# Autodesk Inventor assembly: Кресло простое
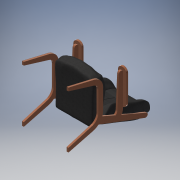
[picture p0: Inventor's stored thumbnail of the model, 180x180]
Saved by Autodesk Inventor 2019 (Build 230136000, 136)
## iProperties
Created: 2018-10-09
Part Number: Кресло простое
Material: Типовые
Document SubType Name: Assembly
Designer: Андреев Н.Л.
Author: Андреев Н.Л.
## Documents named in this file (4)
- C:\Users\andrnl\Documents\Inventor\Мурзин\Кресло простое.iam
- C:\Users\andrnl\Documents\Inventor\Мурзин\Кресло бок.ipt
- C:\Users\andrnl\Documents\Inventor\Мурзин\Upper Seat Cover.ipt
- C:\Users\andrnl\Documents\Inventor\Мурзин\Lower Seat Cushion.ipt
## Components (4 placed, 3 different names)
1. Lower Seat Cushion:1
2. Upper Seat Cover:1
3. Кресло бок:1 — Заподлицо:1, Заподлицо:2, Совмещение:1
4. Кресло бок:2
## Component patterns: (2 elements, first: Кресло бок:1)
## Relationships (3: Flush 2, Mate 1)
- Заподлицо:1 [Flush]: Кресло бок:1
- Заподлицо:2 [Flush] (275 mm): Кресло бок:1
- Совмещение:1 [Mate]: Кресло бок:1
